# Autodesk Inventor assembly: tower
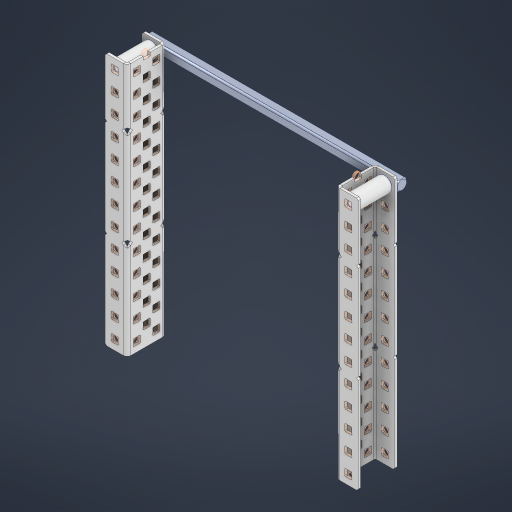
[picture p0: Inventor's stored thumbnail of the model, 512x512]
Saved by Autodesk Inventor 2024 (Build 280153000, 153)
## iProperties
Created: 2023-10-19
Part Number: tower
Document SubType Name: Assembly
Designer: avere
Author: avere
## Documents named in this file (5)
- C:\Users\avere\Documents\rbp_cad\goated_v0.1\catapult\tower.iam
- C:\Users\avere\Documents\rbp_cad\VEX-CAD-Inventor-1.41\Structure\C Channel\Aluminum 1x2x1\Alu C 1x2x1x13.ipt
- C:\Users\avere\Documents\rbp_cad\goated_v0.1\catapult\custom_parts\hs_hardstop\Shaft HS 6.5 in.ipt
- C:\Users\avere\Documents\rbp_cad\goated_v0.1\catapult\custom_parts\hs_hardstop.ipt
- C:\Users\avere\Documents\rbp_cad\hardware\.375 OD Aluminum Spacer 0.875.ipt
## Components (6 placed, 3 different names)
1. Alu C 1x2x1x13:1 — Insert:1, Mate:1, Mate:3, Insert:4
2. Alu C 1x2x1x13:2 — Insert:2, Mate:2, Insert:3, Insert:5
3. Alu C 1x2x1x13:3 — Insert:1, Mate:1, Insert:2, Mate:2
4. Shaft HS 6.5 in:1 — Insert:3, Mate:3
5. .375 OD Aluminum Spacer 0.875:1 — Insert:4
6. .375 OD Aluminum Spacer 0.875:2 — Insert:5
## Relationships (8: Insert 5, Mate 3)
- Insert:1: Alu C 1x2x1x13:1 ↔ Alu C 1x2x1x13:3
- Mate:1: Alu C 1x2x1x13:1 ↔ Alu C 1x2x1x13:3
- Insert:2: Alu C 1x2x1x13:2 ↔ Alu C 1x2x1x13:3
- Mate:2: Alu C 1x2x1x13:2 ↔ Alu C 1x2x1x13:3
- Insert:3: Alu C 1x2x1x13:2 ↔ Shaft HS 6.5 in:1
- Mate:3: Alu C 1x2x1x13:1 ↔ Shaft HS 6.5 in:1
- Insert:4: Alu C 1x2x1x13:1 ↔ .375 OD Aluminum Spacer 0.875:1
- Insert:5: Alu C 1x2x1x13:2 ↔ .375 OD Aluminum Spacer 0.875:2
